# Autodesk Inventor assembly: zlozenie cięcia
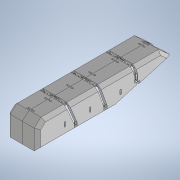
[picture p0: Inventor's stored thumbnail of the model, 180x180]
Saved by Autodesk Inventor 2022.3 (Build 263350000, 350)
## iProperties
Created: 2022-10-28
Part Number: zlozenie cięcia
Document SubType Name: Assembly
Designer: komputer
Author: komputer
## Documents named in this file (15)
- C:\Users\komputer\Desktop\ciecia blotnika\zlozenie cięcia.iam
- C:\Users\komputer\Desktop\ciecia blotnika\blotnik_v3_part_1.ipt
- C:\Users\komputer\Desktop\ciecia blotnika\blotnik_v3_part_2.ipt
- C:\Users\komputer\Desktop\ciecia blotnika\blotnik_v3_part_3.ipt
- C:\Users\komputer\Desktop\ciecia blotnika\blotnik_v3_part_4.ipt
- C:\Users\komputer\Desktop\ciecia blotnika\uchwyt_1.ipt
- C:\Users\komputer\Desktop\ciecia blotnika\uchwyt_2.ipt
- C:\Users\komputer\Desktop\ciecia blotnika\uchwyt_3.ipt
- C:\Users\komputer\Desktop\ciecia blotnika\blotnik_v3_part_1_PRAWA.ipt
- C:\Users\komputer\Desktop\ciecia blotnika\blotnik_v3_part_2_PRAWA.ipt
- C:\Users\komputer\Desktop\ciecia blotnika\blotnik_v3_part_3_PRAWA.ipt
- C:\Users\komputer\Desktop\ciecia blotnika\blotnik_v3_part_4_PRAWA.ipt
- C:\Users\komputer\Desktop\ciecia blotnika\uchwyt_1_PRAWA.ipt
- C:\Users\komputer\Desktop\ciecia blotnika\uchwyt_2_PRAWA.ipt
- C:\Users\komputer\Desktop\ciecia blotnika\uchwyt_3_PRAWA.ipt
## Components (14 placed, 14 different names)
1. blotnik_v3_part_1:1 — Flush:1, Mate:1, Flush:4
2. blotnik_v3_part_2:1 — Flush:1, Flush:2, Mate:1, Mate:2, Flush:4, Flush:5, Mate:5
3. blotnik_v3_part_3:1 — Flush:2, Flush:3, Mate:2, Mate:3, Flush:5, Flush:6, Mate:6
4. blotnik_v3_part_4:1 — Flush:3, Mate:3, Flush:6, Mate:4
5. uchwyt_1:1 — Mate:4
6. uchwyt_2:1 — Mate:6
7. uchwyt_3:1 — Mate:5
8. blotnik_v3_part_1_PRAWA:1 — Flush:7, Mate:7, Flush:8
9. blotnik_v3_part_2_PRAWA:1 — Flush:7, Mate:7, Flush:8, Flush:9, Mate:8, Flush:10, Mate:12
10. blotnik_v3_part_3_PRAWA:1 — Flush:9, Mate:8, Flush:10, Flush:11, Mate:9, Flush:12, Mate:11
11. blotnik_v3_part_4_PRAWA:1 — Flush:11, Mate:9, Flush:12, Mate:10
12. uchwyt_1_PRAWA:1 — Mate:10
13. uchwyt_2_PRAWA:1 — Mate:11
14. uchwyt_3_PRAWA:1 — Mate:12
## Relationships (24: Flush 12, Mate 12)
- Flush:1: blotnik_v3_part_1:1 ↔ blotnik_v3_part_2:1
- Flush:2: blotnik_v3_part_2:1 ↔ blotnik_v3_part_3:1
- Flush:3: blotnik_v3_part_3:1 ↔ blotnik_v3_part_4:1
- Mate:1 (20 mm): blotnik_v3_part_1:1 ↔ blotnik_v3_part_2:1
- Mate:2 (20 mm): blotnik_v3_part_2:1 ↔ blotnik_v3_part_3:1
- Mate:3 (20 mm): blotnik_v3_part_3:1 ↔ blotnik_v3_part_4:1
- Flush:4: blotnik_v3_part_1:1 ↔ blotnik_v3_part_2:1
- Flush:5: blotnik_v3_part_2:1 ↔ blotnik_v3_part_3:1
- Flush:6: blotnik_v3_part_3:1 ↔ blotnik_v3_part_4:1
- Mate:4: blotnik_v3_part_4:1 ↔ uchwyt_1:1
- Mate:5: blotnik_v3_part_2:1 ↔ uchwyt_3:1
- Mate:6: blotnik_v3_part_3:1 ↔ uchwyt_2:1
- Flush:7: blotnik_v3_part_1_PRAWA:1 ↔ blotnik_v3_part_2_PRAWA:1
- Mate:7 (20 mm): blotnik_v3_part_1_PRAWA:1 ↔ blotnik_v3_part_2_PRAWA:1
- Flush:8: blotnik_v3_part_1_PRAWA:1 ↔ blotnik_v3_part_2_PRAWA:1
- Flush:9: blotnik_v3_part_2_PRAWA:1 ↔ blotnik_v3_part_3_PRAWA:1
- Mate:8 (20 mm): blotnik_v3_part_2_PRAWA:1 ↔ blotnik_v3_part_3_PRAWA:1
- Flush:10: blotnik_v3_part_2_PRAWA:1 ↔ blotnik_v3_part_3_PRAWA:1
- Flush:11: blotnik_v3_part_3_PRAWA:1 ↔ blotnik_v3_part_4_PRAWA:1
- Mate:9 (20 mm): blotnik_v3_part_3_PRAWA:1 ↔ blotnik_v3_part_4_PRAWA:1
- Flush:12: blotnik_v3_part_3_PRAWA:1 ↔ blotnik_v3_part_4_PRAWA:1
- Mate:10: blotnik_v3_part_4_PRAWA:1 ↔ uchwyt_1_PRAWA:1
- Mate:11: blotnik_v3_part_3_PRAWA:1 ↔ uchwyt_2_PRAWA:1
- Mate:12: blotnik_v3_part_2_PRAWA:1 ↔ uchwyt_3_PRAWA:1
